# Autodesk Inventor assembly: Drive
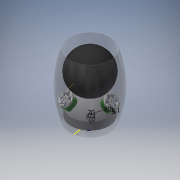
[picture p0: Inventor's stored thumbnail of the model, 180x180]
Saved by Autodesk Inventor 2018.3 (Build 223284000, 284)
## iProperties
Created: 2018-06-30
Part Number: Drive
Material: Generisch
Document SubType Name: Assembly
Designer: JochenAlt
Author: JochenAlt
## Documents named in this file (6)
- D:\Projects\FlowerPot\CAD\Drive.iam
- D:\Projects\FlowerPot\CAD\DriveChain.iam
- D:\Projects\FlowerPot\CAD\Sphere.ipt
- D:\Projects\FlowerPot\CAD\Form.ipt
- D:\Projects\FlowerPot\CAD\FormAxis.ipt
- D:\Projects\FlowerPot\CAD\FormAxisBreak.ipt
## Components (7 placed, 5 different names)
1. Antriebsstrang:1 [sub-assembly] — Passend:1, Passend:3, Passend:5, Tangential:1, Passend:16
2. Antriebsstrang:2 [sub-assembly] — Passend:2, Passend:4, Passend:11, Passend:13, Passend:16
3. Antriebsstrang:3 [sub-assembly] — Passend:1, Passend:2, Passend:3, Passend:4, Passend:12, Passend:13
4. Sphere:1 — Passend:5, Tangential:1
5. Form:1 — Passend:10, Passend:11, Passend:12, Passend:14, Fluchtend:1
6. FormAxis:1 — Passend:14, Fluchtend:1, Passend:15, Fluchtend:2
7. FormAxisBreak:1 — Passend:15, Fluchtend:2
## Relationships (15: Mate 12, Flush 2, Tangent 1)
- Passend:1 [Mate]: Antriebsstrang:1 ↔ Antriebsstrang:3
- Passend:2 [Mate]: Antriebsstrang:2 ↔ Antriebsstrang:3
- Passend:3 [Mate]: Antriebsstrang:1 ↔ Antriebsstrang:3
- Passend:4 [Mate]: Antriebsstrang:2 ↔ Antriebsstrang:3
- Passend:5 [Mate]: Antriebsstrang:1 ↔ Sphere:1
- Tangential:1: Antriebsstrang:1 ↔ Sphere:1
- Passend:10 [Mate]: Form:1
- Passend:11 [Mate]: Antriebsstrang:2 ↔ Form:1
- Passend:12 [Mate]: Antriebsstrang:3 ↔ Form:1
- Passend:13 [Mate]: Antriebsstrang:2 ↔ Antriebsstrang:3
- Passend:14 [Mate]: Form:1 ↔ FormAxis:1
- Fluchtend:1 [Flush]: Form:1 ↔ FormAxis:1
- Passend:15 [Mate]: FormAxis:1 ↔ FormAxisBreak:1
- Fluchtend:2 [Flush]: FormAxis:1 ↔ FormAxisBreak:1
- Passend:16 [Mate]: Antriebsstrang:1 ↔ Antriebsstrang:2
